# Autodesk Inventor assembly: cnc_assembly
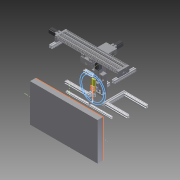
[picture p0: Inventor's stored thumbnail of the model, 180x180]
Saved by Autodesk Inventor 2011 (Build 150239000, 239)
## iProperties
Created: 2012-06-14
Part Number: cnc_assembly
Document SubType Name: Assembly
Designer: labuser
Author: labuser
## Documents named in this file (10)
- C:\Users\labuser\Desktop\cnc_cad\cnc_assembly.iam
- C:\Users\labuser\Desktop\cnc_cad\New XZ_Combo Master.iam
- C:\Users\labuser\Desktop\cnc_cad\z_axis.iam
- C:\Users\labuser\Desktop\cnc_cad\nema_23.ipt
- C:\Users\labuser\Desktop\cnc_cad\head_assembly.iam
- C:\Users\labuser\Desktop\cnc_cad\l_bracket.ipt
- C:\Users\labuser\Documents\GitHub\kinematic_mount\magnet_chuck_redesign\new_assembly.iam
- C:\Users\labuser\Desktop\cnc_cad\8020-25-2525.ipt
- C:\Users\labuser\Desktop\cnc_cad\8020-40-4040-Lite.ipt
- C:\Users\labuser\Desktop\cnc_cad\tv_42i.ipt
## Components (19 placed, 9 different names)
1. New XZ_Combo Master:1 [sub-assembly] — Mate:1, Mate:3, Mate:11, Mate:12, Mate:13, Flush:1, Flush:2, Mate:16, Mate:17
2. z_axis:1 [sub-assembly] — Mate:5, Mate:6, Mate:7, Mate:8, Mate:9, Mate:10, Mate:18, Mate:19
3. nema_23:1 — Mate:3, Mate:16
4. nema_23:2 — Mate:8, Mate:9, Mate:10
5. nema_23:3 — Mate:1, Mate:17
6. head_assembly:1 [sub-assembly] — Mate:5, Mate:6, Mate:7
7. l_bracket:1 — Mate:11, Mate:12, Mate:13, Mate:18, Mate:19
8. new_assembly:1 [sub-assembly]
9. 8020-25-2525:1
10. 8020-25-2525:2
11. 8020-40-4040-Lite:1
12. 8020-40-4040-Lite:2
13. 8020-40-4040-Lite:3
14. 8020-40-4040-Lite:4
15. 8020-40-4040-Lite:5
16. 8020-40-4040-Lite:6
17. 8020-40-4040-Lite:7
18. 8020-40-4040-Lite:8
19. tv_42i:1
## Relationships (17: Mate 15, Flush 2)
- Mate:1: New XZ_Combo Master:1 ↔ nema_23:3
- Mate:3: New XZ_Combo Master:1 ↔ nema_23:1
- Mate:5: z_axis:1 ↔ head_assembly:1
- Mate:6: z_axis:1 ↔ head_assembly:1
- Mate:7: z_axis:1 ↔ head_assembly:1
- Mate:8: z_axis:1 ↔ nema_23:2
- Mate:9: z_axis:1 ↔ nema_23:2
- Mate:10: z_axis:1 ↔ nema_23:2
- Mate:11: New XZ_Combo Master:1 ↔ l_bracket:1
- Mate:12: New XZ_Combo Master:1 ↔ l_bracket:1
- Mate:13: New XZ_Combo Master:1 ↔ l_bracket:1
- Flush:1: New XZ_Combo Master:1
- Flush:2: New XZ_Combo Master:1
- Mate:16: New XZ_Combo Master:1 ↔ nema_23:1
- Mate:17: New XZ_Combo Master:1 ↔ nema_23:3
- Mate:18: z_axis:1 ↔ l_bracket:1
- Mate:19: z_axis:1 ↔ l_bracket:1
